# Autodesk Inventor assembly: subassembly
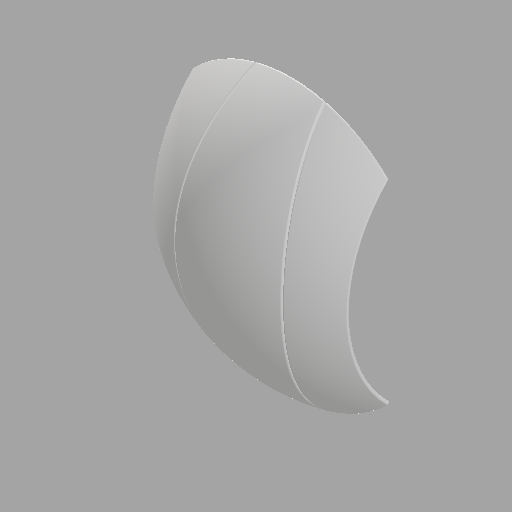
[picture p0: Inventor's stored thumbnail of the model, 512x512]
Saved by Autodesk Inventor 2024 (Build 280153000, 153)
## iProperties
Created: 2024-03-30
Part Number: subassembly
Document SubType Name: Assembly
Designer: Alex
Author: Alex
## Documents named in this file (3)
- C:\Shared\alex-bartella-schoolwork\4z03\Assignment4\subassembly.iam
- C:\Shared\alex-bartella-schoolwork\4z03\Assignment4\middle.ipt
- C:\Shared\alex-bartella-schoolwork\4z03\Assignment4\side.ipt
## Components (3 placed, 2 different names)
1. middle:1 — Flush:1, Mate:1, Flush:2
2. side:1 — Mate:2, Flush:3, Flush:4
3. side:2 — Flush:5, Mate:3, Flush:6
## Relationships (9: Flush 6, Mate 3)
- Flush:1: middle:1
- Mate:1: middle:1
- Flush:2: middle:1
- Mate:2: side:1
- Flush:3: side:1
- Flush:4: side:1
- Flush:5: side:2
- Mate:3: side:2
- Flush:6: side:2
